# Autodesk Inventor assembly: Belt_Unit_Asem
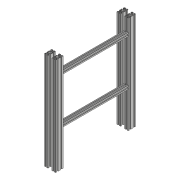
[picture p0: Inventor's stored thumbnail of the model, 180x180]
Saved by Autodesk Inventor 2020.1 (Build 241239000, 239)
## iProperties
Created: 2020-06-08
Part Number: Belt_Unit_Asem
Document SubType Name: Assembly
Designer: ken113
Author: ken113
## Documents named in this file (3)
- D:\ken113\Documents\GitHub\Cheap_Belt_Printer\Model\Asem\Belt_Unit_Asem.iam
- D:\ken113\Documents\GitHub\Cheap_Belt_Printer\Model\Parts\MISUMI\HFS5-2020-340_Autodesk_Inventor_2020_20201001\HFS5-2020-340.ipt
- D:\ken113\Documents\GitHub\Cheap_Belt_Printer\Model\Parts\MISUMI\HFS5-2040-510_Autodesk_Inventor_2020_20201006\HFS5-2040-510.ipt
## Components (6 placed, 2 different names)
1. HFS5-2040-510:1 — 対称度:1, フラッシュ:15, フラッシュ:16, メイト:9
2. HFS5-2040-510:2 — 対称度:1, フラッシュ:14
3. HFS5-2020-340:2 — Flush:10
4. HFS5-2020-340:3 — Flush:10
5. HFS5-2040-510:3 — フラッシュ:12, フラッシュ:13, フラッシュ:14
6. HFS5-2040-510:4 — フラッシュ:12, フラッシュ:13, フラッシュ:15, フラッシュ:16, メイト:9
## Relationships (16: Flush 10, Mate 5, Symmetry 1)
- [Flush]: HFS5-2040-510:1 ↔ HFS5-2040-510:2
- [Flush]: HFS5-2040-510:1 ↔ HFS5-2040-510:2
- [Mate] (340 mm): HFS5-2040-510:1 ↔ HFS5-2040-510:2
- [Mate]: HFS5-2040-510:2 ↔ HFS5-2020-340:3
- [Mate]: HFS5-2040-510:2 ↔ HFS5-2020-340:2
- [Flush]: HFS5-2040-510:1 ↔ HFS5-2020-340:3
- Flush:10: HFS5-2020-340:2 ↔ HFS5-2020-340:3
- 対称度:1 [Symmetry]: HFS5-2040-510:1 ↔ HFS5-2040-510:2
- フラッシュ:11 [Flush]
- メイト:8 [Mate]
- フラッシュ:12 [Flush]: HFS5-2040-510:3 ↔ HFS5-2040-510:4
- フラッシュ:13 [Flush]: HFS5-2040-510:3 ↔ HFS5-2040-510:4
- フラッシュ:14 [Flush]: HFS5-2040-510:2 ↔ HFS5-2040-510:3
- フラッシュ:15 [Flush]: HFS5-2040-510:1 ↔ HFS5-2040-510:4
- フラッシュ:16 [Flush]: HFS5-2040-510:1 ↔ HFS5-2040-510:4
- メイト:9 [Mate] (20 mm): HFS5-2040-510:1 ↔ HFS5-2040-510:4
